# Autodesk Inventor assembly: Mock Module PCB
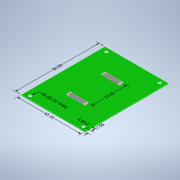
[picture p0: Inventor's stored thumbnail of the model, 180x180]
Saved by Autodesk Inventor 2022 (Build 260153000, 153)
## iProperties
Created: 2021-07-19
Part Number: Mock Module PCB
Document SubType Name: Assembly
Designer: Caleb
Author: Caleb
## Documents named in this file (3)
- C:\Users\Caleb\Desktop\nebraska-silicon-lab\Hardware\ETL\modules\tamale\Mock Module PCB - V2p1.iam
- C:\Users\Caleb\Desktop\nebraska-silicon-lab\Hardware\ETL\ETL-SH-Design\3D-model\K3D-WP7B-S050VA1-V3_JAE_Proprietary v1_14.iam
- C:\Users\Caleb\Desktop\nebraska-silicon-lab\Hardware\ETL\modules\tamale\Mock Module PCB - V2p1.ipt
## Components (3 placed, 2 different names)
1. Mock Module PCB - V2p1:1 — Mate:1, Mate:2, Flush:4, Flush:6
2. K3D-WP7B-S050VA1-V3_JAE_Proprietary v1_14:1 [sub-assembly] — Mate:1, Flush:3, Flush:5
3. K3D-WP7B-S050VA1-V3_JAE_Proprietary v1_14:2 [sub-assembly] — Mate:2, Flush:3, Flush:4, Flush:5, Flush:6
## Relationships (6: Flush 4, Mate 2)
- Mate:1: Mock Module PCB - V2p1:1 ↔ K3D-WP7B-S050VA1-V3_JAE_Proprietary v1_14:1
- Mate:2: Mock Module PCB - V2p1:1 ↔ K3D-WP7B-S050VA1-V3_JAE_Proprietary v1_14:2
- Flush:3 (23.531 mm): K3D-WP7B-S050VA1-V3_JAE_Proprietary v1_14:1 ↔ K3D-WP7B-S050VA1-V3_JAE_Proprietary v1_14:2
- Flush:4 (15.2945 mm): Mock Module PCB - V2p1:1 ↔ K3D-WP7B-S050VA1-V3_JAE_Proprietary v1_14:2
- Flush:5: K3D-WP7B-S050VA1-V3_JAE_Proprietary v1_14:1 ↔ K3D-WP7B-S050VA1-V3_JAE_Proprietary v1_14:2
- Flush:6 (15.307 mm): Mock Module PCB - V2p1:1 ↔ K3D-WP7B-S050VA1-V3_JAE_Proprietary v1_14:2
